# Autodesk Inventor assembly: CIM Motor
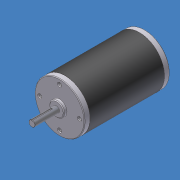
[picture p0: Inventor's stored thumbnail of the model, 180x180]
Saved by Autodesk Inventor 2012 (Build 160160000, 160)
## iProperties
Shininess: 64.0
Length Units: 11272
Angle Units: 11279
Time Units: 11290
Mass Units: 11286
Length Display Precision: 3
Angle Display Precision: 2
Compacted: True
Part Number: CIM Motor
Document SubType Name: Assembly
Created: 2006-01-16
Designer: Ed Sparks
Density: 0.0
Volumn: 0.0
Area: 0.0
PropertySet Name: Model Information
Control State: 0
Master: False
Checked Out: False
Author: Ed Sparks
## Documents named in this file (4)
- C:\Users\Bryce\Dropbox\Inventor Design Project Files\Independent Swerves\Imported Components\CIM Motor.iam
- C:\Users\Bryce\Dropbox\Inventor Design Project Files\Independent Swerves\Imported Components\CIM motor.ipt
- C:\Users\Bryce\Dropbox\Inventor Design Project Files\Independent Swerves\Imported Components\10-24 UNC x 4_ Phillips Pan Head.ipt
- C:\Household Files\Bruce Work\Inventor Projects\Inventor library\Motors\CIM Motor Assy\Phillips Pan Head Machine Screw Inch.ipt
## Components (3 placed, 2 different names)
1. CIM motor:1 — Mate:1, Mate:2
2. 10-24 UNC x 4_ Phillips Pan Head:1 — Mate:1, Mate:2
3. 10-24 UNC x 4_ Phillips Pan Head:2
## Component patterns: (2 elements, first: 10-24 UNC x 4_ Phillips Pan Head:1)
## Relationships (2: Mate 2)
- Mate:1: CIM motor:1 ↔ 10-24 UNC x 4_ Phillips Pan Head:1
- Mate:2: CIM motor:1 ↔ 10-24 UNC x 4_ Phillips Pan Head:1
